# Autodesk Inventor assembly: glassMitSchutz_MIR
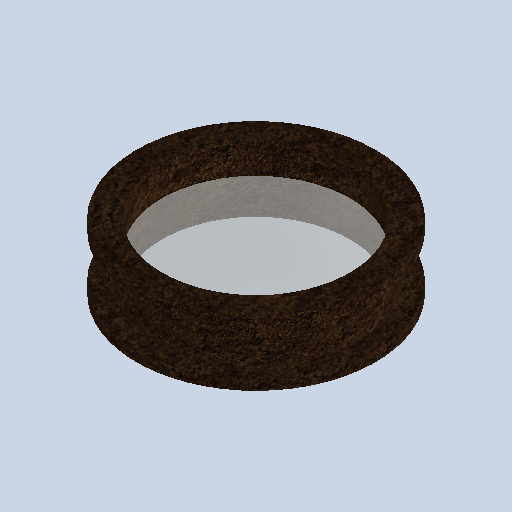
[picture p0: Inventor's stored thumbnail of the model, 512x512]
Saved by Autodesk Inventor 2025.1 (Build 291241000, 241)
## iProperties
Created: 2024-08-07
Part Number: glassMitSchutz_MIR
Document SubType Name: Assembly
Designer: ffogue
Author: ffogue
## Documents named in this file (3)
- C:\Users\ffogue\Documents\Inventor\BrandschutzTuer\glassMitSchutz_MIR.iam
- C:\Users\ffogue\Documents\Inventor\BrandschutzTuer\glassSchutz_MIR.ipt
- C:\Users\ffogue\Documents\Inventor\BrandschutzTuer\glass_MIR.ipt
## Components (3 placed, 2 different names)
1. glassSchutz_MIR:1 — Insert:1
2. glass_MIR:1 — Insert:1, Insert:2
3. glassSchutz_MIR:2 — Insert:2
## Relationships (2: Insert 2)
- Insert:1: glassSchutz_MIR:1 ↔ glass_MIR:1
- Insert:2: glass_MIR:1 ↔ glassSchutz_MIR:2
